# Autodesk Inventor assembly: steelSlides
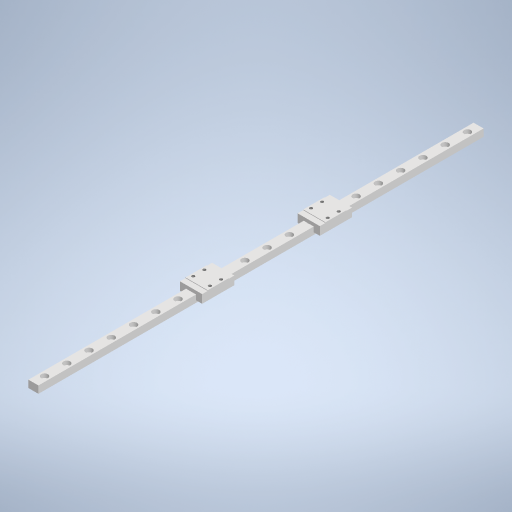
[picture p0: Inventor's stored thumbnail of the model, 512x512]
Saved by Autodesk Inventor 2023 (Build 270158000, 158)
## iProperties
Created: 2022-09-16
Part Number: steelSlides
Document SubType Name: Assembly
Designer: deli
Author: deli
## Documents named in this file (3)
- C:\Users\deli\OneDrive - Eastside Preparatory School\FTC\8103-power-play\CAD\steelSlides.iam
- C:\Users\deli\OneDrive - Eastside Preparatory School\FTC\8103-power-play\CAD\Rail.ipt
- C:\Users\deli\OneDrive - Eastside Preparatory School\FTC\8103-power-play\CAD\Carrige.ipt
## Components (3 placed, 2 different names)
1. Rail:1 — Mate:1, Mate:2, Mate:3, Mate:4
2. Carrige:1 — Mate:1, Mate:2
3. Carrige:2 — Mate:3, Mate:4
## Relationships (4: Mate 4)
- Mate:1: Rail:1 ↔ Carrige:1
- Mate:2: Rail:1 ↔ Carrige:1
- Mate:3: Rail:1 ↔ Carrige:2
- Mate:4: Rail:1 ↔ Carrige:2
